# Autodesk Inventor assembly: COSI_MINI_V1
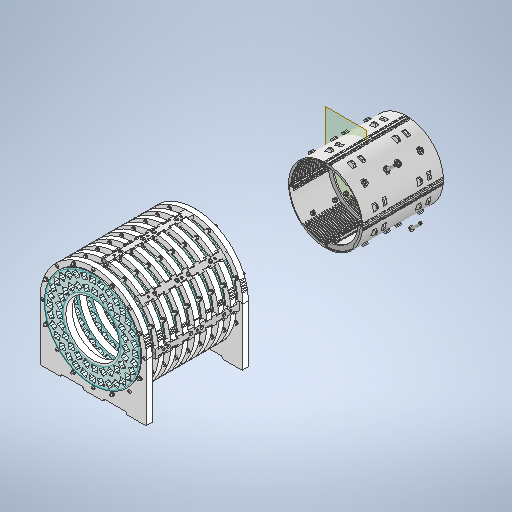
[picture p0: Inventor's stored thumbnail of the model, 512x512]
Saved by Autodesk Inventor 2025.2 (Build 292293000, 293)
## iProperties
Created: 2023-07-27
Part Number: COSI_MINI_V1
Document SubType Name: Assembly
Designer: Joshua Harper
Author: Joshua Harper
## Documents named in this file (17)
- C:\Users\Carla Fernandez\Documents\GitHub\OSII_MINI_V2\CAD MODELS\COSI_MINI_V2.iam
- C:\Users\Carla Fernandez\Documents\GitHub\OSII_MINI_V2\CAD MODELS\Ring_0.ipt
- C:\Users\Carla Fernandez\Documents\GitHub\OSII_MINI_V2\CAD MODELS\Ring_1.ipt
- C:\Users\Carla Fernandez\Documents\GitHub\OSII_MINI_V2\CAD MODELS\Ring_2.ipt
- C:\Users\Carla Fernandez\Documents\GitHub\OSII_MINI_V2\CAD MODELS\Ring_3.ipt
- C:\Users\Carla Fernandez\Documents\GitHub\OSII_MINI_V2\CAD MODELS\Ring_4.ipt
- C:\Users\Carla Fernandez\Documents\GitHub\OSII_MINI_V2\CAD MODELS\M4_threaded_brass.ipt
- C:\Users\Carla Fernandez\Documents\GitHub\OSII_MINI_V2\CAD MODELS\Locating_bar_V2.ipt
- C:\Users\Carla Fernandez\Documents\GitHub\OSII_MINI_V2\CAD MODELS\93187A150_NO THREADS_Brass Thin Hex Nut.ipt
- C:\Users\Carla Fernandez\Documents\GitHub\OSII_MINI_V2\CAD MODELS\98691A114_General Purpose Brass Washer.ipt
- C:\Users\Carla Fernandez\Documents\GitHub\OSII_MINI_V2\CAD MODELS\94500A283_NO THREADS_316 Stainless Steel Button Head Hex Drive Screws.ipt
- C:\Users\Carla Fernandez\Documents\GitHub\OSII_MINI_V2\CAD MODELS\94500A283_NO THREADS_316 Stainless Steel Button Head Hex Drive Screws_MIR.ipt
- C:\Users\Carla Fernandez\Documents\GitHub\OSII_MINI_V2\CAD MODELS\Lid_A.ipt
- C:\Users\Carla Fernandez\Documents\GitHub\OSII_MINI_V2\CAD MODELS\Lid_B.ipt
- C:\Users\Carla Fernandez\Documents\GitHub\OSII_MINI_V2\CAD MODELS\Shim_Assem_V4.iam
- C:\Users\Carla Fernandez\Documents\GitHub\OSII_MINI_V2\CAD MODELS\shim_cartridge_V3.ipt
- C:\Users\Carla Fernandez\Documents\GitHub\OSII_MINI_V2\CAD MODELS\shim_peg_V3.ipt
## Components (341 placed, 16 different names)
1. Ring_0:1 — Mate:4, Mate:5, Mate:16, Mate:37, Mate:39, Mate:43, Mate:48, Mate:51, Mate:54, Mate:55, Mate:57, Mate:70, Mate:71, Flush:3, Flush:4, Flush:5, Flush:6
2. Ring_1:1 — Mate:5, Mate:17, Flush:3
3. Ring_1:2 — Mate:3, Mate:4, Mate:10, Mate:16
4. Ring_2:1 — Mate:6, Mate:17, Flush:4
5. Ring_2:2 — Mate:2, Mate:3, Mate:9, Mate:10
6. Ring_3:1 — Mate:6, Mate:7, Flush:5
7. Ring_3:2 — Mate:1, Mate:2, Mate:8, Mate:9, Mate:36
8. Ring_4:1 — Mate:7, Flush:6, Mate:72, Mate:73
9. Ring_4:2 — Mate:1, Mate:8, Mate:26, Mate:35, Mate:62, Mate:63, Mate:68, Mate:76
10. Locating_bar_V2:1 — Mate:35, Mate:36, Mate:69
11. Locating_bar_V2:2 — Mate:37, Mate:39, Mate:76
12. Locating_bar_V2:3
13. Locating_bar_V2:4 — Mate:54
14. Locating_bar_V2:5 — Mate:43
15. Locating_bar_V2:6 — Mate:55, Mate:57
16. Locating_bar_V2:7 — Mate:51
17. Locating_bar_V2:8 — Mate:48
18. Shim_Assem_V4:1 [sub-assembly] — Mate:77, Mate:78, Mate:79, Mate:80, Mate:81
19. shim_cartridge_V3:1 — Mate:79, Mate:80, Mate:81
20. shim_peg_V3:1 — Mate:77, Mate:78
21. 94500A283_NO THREADS_316 Stainless Steel Button Head Hex Drive Screws:1 — Mate:68, Mate:69
22. 94500A283_NO THREADS_316 Stainless Steel Button Head Hex Drive Screws:2
23. 94500A283_NO THREADS_316 Stainless Steel Button Head Hex Drive Screws:3
24. 94500A283_NO THREADS_316 Stainless Steel Button Head Hex Drive Screws:4
25. 94500A283_NO THREADS_316 Stainless Steel Button Head Hex Drive Screws:5
26. 94500A283_NO THREADS_316 Stainless Steel Button Head Hex Drive Screws:6
27. 94500A283_NO THREADS_316 Stainless Steel Button Head Hex Drive Screws:7
28. 94500A283_NO THREADS_316 Stainless Steel Button Head Hex Drive Screws:8
29. Lid_A:1 — Mate:70, Mate:71
30. Lid_A:2
31. Lid_A:3
32. Lid_A:4
33. Lid_A:5
34. Lid_A:6
35. Lid_A:7
36. Lid_B:1
37. Lid_B:2
38. 94500A283_NO THREADS_316 Stainless Steel Button Head Hex Drive Screws_MIR:1 — Mate:72, Mate:73
39. 94500A283_NO THREADS_316 Stainless Steel Button Head Hex Drive Screws_MIR:2
40. 94500A283_NO THREADS_316 Stainless Steel Button Head Hex Drive Screws_MIR:3
41. 94500A283_NO THREADS_316 Stainless Steel Button Head Hex Drive Screws_MIR:4
42. 94500A283_NO THREADS_316 Stainless Steel Button Head Hex Drive Screws_MIR:5
43. 94500A283_NO THREADS_316 Stainless Steel Button Head Hex Drive Screws_MIR:6
44. 94500A283_NO THREADS_316 Stainless Steel Button Head Hex Drive Screws_MIR:7
45. 94500A283_NO THREADS_316 Stainless Steel Button Head Hex Drive Screws_MIR:8
46. M4_threaded_brass:1 — Mate:26
47. M4_threaded_brass:2
48. M4_threaded_brass:3
49. M4_threaded_brass:4
50. M4_threaded_brass:5
51. M4_threaded_brass:6
52. M4_threaded_brass:7
53. M4_threaded_brass:8
54. 93187A150_NO THREADS_Brass Thin Hex Nut:1 — Mate:67
55. 93187A150_NO THREADS_Brass Thin Hex Nut:2 — Mate:66
56. 98691A114_General Purpose Brass Washer:1 — Mate:62, Mate:67
57. 98691A114_General Purpose Brass Washer:2 — Mate:63, Mate:66
58. 93187A150_NO THREADS_Brass Thin Hex Nut:3
59. 93187A150_NO THREADS_Brass Thin Hex Nut:4
60. 98691A114_General Purpose Brass Washer:3
61. 98691A114_General Purpose Brass Washer:4
62. 93187A150_NO THREADS_Brass Thin Hex Nut:5
63. 93187A150_NO THREADS_Brass Thin Hex Nut:6
64. 98691A114_General Purpose Brass Washer:5
65. 98691A114_General Purpose Brass Washer:6
66. 93187A150_NO THREADS_Brass Thin Hex Nut:7
67. 93187A150_NO THREADS_Brass Thin Hex Nut:8
68. 98691A114_General Purpose Brass Washer:7
69. 98691A114_General Purpose Brass Washer:8
70. 93187A150_NO THREADS_Brass Thin Hex Nut:9
71. 93187A150_NO THREADS_Brass Thin Hex Nut:10
72. 98691A114_General Purpose Brass Washer:9
73. 98691A114_General Purpose Brass Washer:10
74. 93187A150_NO THREADS_Brass Thin Hex Nut:11
75. 93187A150_NO THREADS_Brass Thin Hex Nut:12
76. 98691A114_General Purpose Brass Washer:11
77. 98691A114_General Purpose Brass Washer:12
78. 93187A150_NO THREADS_Brass Thin Hex Nut:13
79. 93187A150_NO THREADS_Brass Thin Hex Nut:14
80. 98691A114_General Purpose Brass Washer:13
81. 98691A114_General Purpose Brass Washer:14
82. 93187A150_NO THREADS_Brass Thin Hex Nut:15
83. 93187A150_NO THREADS_Brass Thin Hex Nut:16
84. 98691A114_General Purpose Brass Washer:15
85. 98691A114_General Purpose Brass Washer:16
86. 93187A150_NO THREADS_Brass Thin Hex Nut:17
87. 93187A150_NO THREADS_Brass Thin Hex Nut:18
88. 98691A114_General Purpose Brass Washer:17
89. 98691A114_General Purpose Brass Washer:18
90. 93187A150_NO THREADS_Brass Thin Hex Nut:19
91. 93187A150_NO THREADS_Brass Thin Hex Nut:20
92. 98691A114_General Purpose Brass Washer:19
93. 98691A114_General Purpose Brass Washer:20
94. 93187A150_NO THREADS_Brass Thin Hex Nut:21
95. 93187A150_NO THREADS_Brass Thin Hex Nut:22
96. 98691A114_General Purpose Brass Washer:21
97. 98691A114_General Purpose Brass Washer:22
98. 93187A150_NO THREADS_Brass Thin Hex Nut:23
99. 93187A150_NO THREADS_Brass Thin Hex Nut:24
100. 98691A114_General Purpose Brass Washer:23
101. 98691A114_General Purpose Brass Washer:24
102. 93187A150_NO THREADS_Brass Thin Hex Nut:25
103. 93187A150_NO THREADS_Brass Thin Hex Nut:26
104. 98691A114_General Purpose Brass Washer:25
105. 98691A114_General Purpose Brass Washer:26
106. 93187A150_NO THREADS_Brass Thin Hex Nut:27
107. 93187A150_NO THREADS_Brass Thin Hex Nut:28
108. 98691A114_General Purpose Brass Washer:27
109. 98691A114_General Purpose Brass Washer:28
110. 93187A150_NO THREADS_Brass Thin Hex Nut:29
111. 93187A150_NO THREADS_Brass Thin Hex Nut:30
112. 98691A114_General Purpose Brass Washer:29
113. 98691A114_General Purpose Brass Washer:30
114. 93187A150_NO THREADS_Brass Thin Hex Nut:31
115. 93187A150_NO THREADS_Brass Thin Hex Nut:32
116. 98691A114_General Purpose Brass Washer:31
117. 98691A114_General Purpose Brass Washer:32
118. 93187A150_NO THREADS_Brass Thin Hex Nut:33
119. 93187A150_NO THREADS_Brass Thin Hex Nut:34
120. 98691A114_General Purpose Brass Washer:33
121. 98691A114_General Purpose Brass Washer:34
122. 93187A150_NO THREADS_Brass Thin Hex Nut:35
123. 93187A150_NO THREADS_Brass Thin Hex Nut:36
124. 98691A114_General Purpose Brass Washer:35
125. 98691A114_General Purpose Brass Washer:36
126. 93187A150_NO THREADS_Brass Thin Hex Nut:37
127. 93187A150_NO THREADS_Brass Thin Hex Nut:38
128. 98691A114_General Purpose Brass Washer:37
129. 98691A114_General Purpose Brass Washer:38
130. 93187A150_NO THREADS_Brass Thin Hex Nut:39
131. 93187A150_NO THREADS_Brass Thin Hex Nut:40
132. 98691A114_General Purpose Brass Washer:39
133. 98691A114_General Purpose Brass Washer:40
134. 93187A150_NO THREADS_Brass Thin Hex Nut:41
135. 93187A150_NO THREADS_Brass Thin Hex Nut:42
136. 98691A114_General Purpose Brass Washer:41
137. 98691A114_General Purpose Brass Washer:42
138. 93187A150_NO THREADS_Brass Thin Hex Nut:43
139. 93187A150_NO THREADS_Brass Thin Hex Nut:44
140. 98691A114_General Purpose Brass Washer:43
141. 98691A114_General Purpose Brass Washer:44
142. 93187A150_NO THREADS_Brass Thin Hex Nut:45
143. 93187A150_NO THREADS_Brass Thin Hex Nut:46
144. 98691A114_General Purpose Brass Washer:45
145. 98691A114_General Purpose Brass Washer:46
146. 93187A150_NO THREADS_Brass Thin Hex Nut:47
147. 93187A150_NO THREADS_Brass Thin Hex Nut:48
148. 98691A114_General Purpose Brass Washer:47
149. 98691A114_General Purpose Brass Washer:48
150. 93187A150_NO THREADS_Brass Thin Hex Nut:49
151. 93187A150_NO THREADS_Brass Thin Hex Nut:50
152. 98691A114_General Purpose Brass Washer:49
153. 98691A114_General Purpose Brass Washer:50
154. 93187A150_NO THREADS_Brass Thin Hex Nut:51
155. 93187A150_NO THREADS_Brass Thin Hex Nut:52
156. 98691A114_General Purpose Brass Washer:51
157. 98691A114_General Purpose Brass Washer:52
158. 93187A150_NO THREADS_Brass Thin Hex Nut:53
159. 93187A150_NO THREADS_Brass Thin Hex Nut:54
160. 98691A114_General Purpose Brass Washer:53
161. 98691A114_General Purpose Brass Washer:54
162. 93187A150_NO THREADS_Brass Thin Hex Nut:55
163. 93187A150_NO THREADS_Brass Thin Hex Nut:56
164. 98691A114_General Purpose Brass Washer:55
165. 98691A114_General Purpose Brass Washer:56
166. 93187A150_NO THREADS_Brass Thin Hex Nut:57
167. 93187A150_NO THREADS_Brass Thin Hex Nut:58
168. 98691A114_General Purpose Brass Washer:57
169. 98691A114_General Purpose Brass Washer:58
170. 93187A150_NO THREADS_Brass Thin Hex Nut:59
171. 93187A150_NO THREADS_Brass Thin Hex Nut:60
172. 98691A114_General Purpose Brass Washer:59
173. 98691A114_General Purpose Brass Washer:60
174. 93187A150_NO THREADS_Brass Thin Hex Nut:61
175. 93187A150_NO THREADS_Brass Thin Hex Nut:62
176. 98691A114_General Purpose Brass Washer:61
177. 98691A114_General Purpose Brass Washer:62
178. 93187A150_NO THREADS_Brass Thin Hex Nut:63
179. 93187A150_NO THREADS_Brass Thin Hex Nut:64
180. 98691A114_General Purpose Brass Washer:63
181. 98691A114_General Purpose Brass Washer:64
182. 93187A150_NO THREADS_Brass Thin Hex Nut:65
183. 93187A150_NO THREADS_Brass Thin Hex Nut:66
184. 98691A114_General Purpose Brass Washer:65
185. 98691A114_General Purpose Brass Washer:66
186. 93187A150_NO THREADS_Brass Thin Hex Nut:67
187. 93187A150_NO THREADS_Brass Thin Hex Nut:68
188. 98691A114_General Purpose Brass Washer:67
189. 98691A114_General Purpose Brass Washer:68
190. 93187A150_NO THREADS_Brass Thin Hex Nut:69
191. 93187A150_NO THREADS_Brass Thin Hex Nut:70
192. 98691A114_General Purpose Brass Washer:69
193. 98691A114_General Purpose Brass Washer:70
194. 93187A150_NO THREADS_Brass Thin Hex Nut:71
195. 93187A150_NO THREADS_Brass Thin Hex Nut:72
196. 98691A114_General Purpose Brass Washer:71
197. 98691A114_General Purpose Brass Washer:72
198. 93187A150_NO THREADS_Brass Thin Hex Nut:73
199. 93187A150_NO THREADS_Brass Thin Hex Nut:74
200. 98691A114_General Purpose Brass Washer:73
201. 98691A114_General Purpose Brass Washer:74
202. 93187A150_NO THREADS_Brass Thin Hex Nut:75
203. 93187A150_NO THREADS_Brass Thin Hex Nut:76
204. 98691A114_General Purpose Brass Washer:75
205. 98691A114_General Purpose Brass Washer:76
206. 93187A150_NO THREADS_Brass Thin Hex Nut:77
207. 93187A150_NO THREADS_Brass Thin Hex Nut:78
208. 98691A114_General Purpose Brass Washer:77
209. 98691A114_General Purpose Brass Washer:78
210. 93187A150_NO THREADS_Brass Thin Hex Nut:79
211. 93187A150_NO THREADS_Brass Thin Hex Nut:80
212. 98691A114_General Purpose Brass Washer:79
213. 98691A114_General Purpose Brass Washer:80
214. 93187A150_NO THREADS_Brass Thin Hex Nut:81
215. 93187A150_NO THREADS_Brass Thin Hex Nut:82
216. 98691A114_General Purpose Brass Washer:81
217. 98691A114_General Purpose Brass Washer:82
218. 93187A150_NO THREADS_Brass Thin Hex Nut:83
219. 93187A150_NO THREADS_Brass Thin Hex Nut:84
220. 98691A114_General Purpose Brass Washer:83
221. 98691A114_General Purpose Brass Washer:84
222. 93187A150_NO THREADS_Brass Thin Hex Nut:85
223. 93187A150_NO THREADS_Brass Thin Hex Nut:86
224. 98691A114_General Purpose Brass Washer:85
225. 98691A114_General Purpose Brass Washer:86
226. 93187A150_NO THREADS_Brass Thin Hex Nut:87
227. 93187A150_NO THREADS_Brass Thin Hex Nut:88
228. 98691A114_General Purpose Brass Washer:87
229. 98691A114_General Purpose Brass Washer:88
230. 93187A150_NO THREADS_Brass Thin Hex Nut:89
231. 93187A150_NO THREADS_Brass Thin Hex Nut:90
232. 98691A114_General Purpose Brass Washer:89
233. 98691A114_General Purpose Brass Washer:90
234. 93187A150_NO THREADS_Brass Thin Hex Nut:91
235. 93187A150_NO THREADS_Brass Thin Hex Nut:92
236. 98691A114_General Purpose Brass Washer:91
237. 98691A114_General Purpose Brass Washer:92
238. 93187A150_NO THREADS_Brass Thin Hex Nut:93
239. 93187A150_NO THREADS_Brass Thin Hex Nut:94
240. 98691A114_General Purpose Brass Washer:93
241. 98691A114_General Purpose Brass Washer:94
242. 93187A150_NO THREADS_Brass Thin Hex Nut:95
243. 93187A150_NO THREADS_Brass Thin Hex Nut:96
244. 98691A114_General Purpose Brass Washer:95
245. 98691A114_General Purpose Brass Washer:96
246. 93187A150_NO THREADS_Brass Thin Hex Nut:97
247. 93187A150_NO THREADS_Brass Thin Hex Nut:98
248. 98691A114_General Purpose Brass Washer:97
249. 98691A114_General Purpose Brass Washer:98
250. 93187A150_NO THREADS_Brass Thin Hex Nut:99
251. 93187A150_NO THREADS_Brass Thin Hex Nut:100
252. 98691A114_General Purpose Brass Washer:99
253. 98691A114_General Purpose Brass Washer:100
254. 93187A150_NO THREADS_Brass Thin Hex Nut:101
255. 93187A150_NO THREADS_Brass Thin Hex Nut:102
256. 98691A114_General Purpose Brass Washer:101
257. 98691A114_General Purpose Brass Washer:102
258. 93187A150_NO THREADS_Brass Thin Hex Nut:103
259. 93187A150_NO THREADS_Brass Thin Hex Nut:104
260. 98691A114_General Purpose Brass Washer:103
261. 98691A114_General Purpose Brass Washer:104
262. 93187A150_NO THREADS_Brass Thin Hex Nut:105
263. 93187A150_NO THREADS_Brass Thin Hex Nut:106
264. 98691A114_General Purpose Brass Washer:105
265. 98691A114_General Purpose Brass Washer:106
266. 93187A150_NO THREADS_Brass Thin Hex Nut:107
267. 93187A150_NO THREADS_Brass Thin Hex Nut:108
268. 98691A114_General Purpose Brass Washer:107
269. 98691A114_General Purpose Brass Washer:108
270. 93187A150_NO THREADS_Brass Thin Hex Nut:109
271. 93187A150_NO THREADS_Brass Thin Hex Nut:110
272. 98691A114_General Purpose Brass Washer:109
273. 98691A114_General Purpose Brass Washer:110
274. 93187A150_NO THREADS_Brass Thin Hex Nut:111
275. 93187A150_NO THREADS_Brass Thin Hex Nut:112
276. 98691A114_General Purpose Brass Washer:111
277. 98691A114_General Purpose Brass Washer:112
278. 93187A150_NO THREADS_Brass Thin Hex Nut:113
279. 93187A150_NO THREADS_Brass Thin Hex Nut:114
280. 98691A114_General Purpose Brass Washer:113
281. 98691A114_General Purpose Brass Washer:114
282. 93187A150_NO THREADS_Brass Thin Hex Nut:115
283. 93187A150_NO THREADS_Brass Thin Hex Nut:116
284. 98691A114_General Purpose Brass Washer:115
285. 98691A114_General Purpose Brass Washer:116
286. 93187A150_NO THREADS_Brass Thin Hex Nut:117
287. 93187A150_NO THREADS_Brass Thin Hex Nut:118
288. 98691A114_General Purpose Brass Washer:117
289. 98691A114_General Purpose Brass Washer:118
290. 93187A150_NO THREADS_Brass Thin Hex Nut:119
291. 93187A150_NO THREADS_Brass Thin Hex Nut:120
292. 98691A114_General Purpose Brass Washer:119
293. 98691A114_General Purpose Brass Washer:120
294. 93187A150_NO THREADS_Brass Thin Hex Nut:121
295. 93187A150_NO THREADS_Brass Thin Hex Nut:122
296. 98691A114_General Purpose Brass Washer:121
297. 98691A114_General Purpose Brass Washer:122
298. 93187A150_NO THREADS_Brass Thin Hex Nut:123
299. 93187A150_NO THREADS_Brass Thin Hex Nut:124
300. 98691A114_General Purpose Brass Washer:123
301. 98691A114_General Purpose Brass Washer:124
302. 93187A150_NO THREADS_Brass Thin Hex Nut:125
303. 93187A150_NO THREADS_Brass Thin Hex Nut:126
304. 98691A114_General Purpose Brass Washer:125
305. 98691A114_General Purpose Brass Washer:126
306. 93187A150_NO THREADS_Brass Thin Hex Nut:127
307. 93187A150_NO THREADS_Brass Thin Hex Nut:128
308. 98691A114_General Purpose Brass Washer:127
309. 98691A114_General Purpose Brass Washer:128
310. 93187A150_NO THREADS_Brass Thin Hex Nut:129
311. 93187A150_NO THREADS_Brass Thin Hex Nut:130
312. 98691A114_General Purpose Brass Washer:129
313. 98691A114_General Purpose Brass Washer:130
314. 93187A150_NO THREADS_Brass Thin Hex Nut:131
315. 93187A150_NO THREADS_Brass Thin Hex Nut:132
316. 98691A114_General Purpose Brass Washer:131
317. 98691A114_General Purpose Brass Washer:132
318. 93187A150_NO THREADS_Brass Thin Hex Nut:133
319. 93187A150_NO THREADS_Brass Thin Hex Nut:134
320. 98691A114_General Purpose Brass Washer:133
321. 98691A114_General Purpose Brass Washer:134
322. 93187A150_NO THREADS_Brass Thin Hex Nut:135
323. 93187A150_NO THREADS_Brass Thin Hex Nut:136
324. 98691A114_General Purpose Brass Washer:135
325. 98691A114_General Purpose Brass Washer:136
326. 93187A150_NO THREADS_Brass Thin Hex Nut:137
327. 93187A150_NO THREADS_Brass Thin Hex Nut:138
328. 98691A114_General Purpose Brass Washer:137
329. 98691A114_General Purpose Brass Washer:138
330. 93187A150_NO THREADS_Brass Thin Hex Nut:139
331. 93187A150_NO THREADS_Brass Thin Hex Nut:140
332. 98691A114_General Purpose Brass Washer:139
333. 98691A114_General Purpose Brass Washer:140
334. 93187A150_NO THREADS_Brass Thin Hex Nut:141
335. 93187A150_NO THREADS_Brass Thin Hex Nut:142
336. 98691A114_General Purpose Brass Washer:141
337. 98691A114_General Purpose Brass Washer:142
338. 93187A150_NO THREADS_Brass Thin Hex Nut:143
339. 93187A150_NO THREADS_Brass Thin Hex Nut:144
340. 98691A114_General Purpose Brass Washer:143
341. 98691A114_General Purpose Brass Washer:144
## Component patterns: (8 elements), (8 elements, first: 94500A283_NO THREADS_316 Stainless Steel Button Head Hex Drive Screws:1), (7 elements, first: Lid_A:1), (2 elements, first: Lid_B:1), (8 elements, first: 94500A283_NO THREADS_316 Stainless Steel Button Head Hex Drive Screws_MIR:1), (8 elements, first: M4_threaded_brass:1), (9 elements, first: 93187A150_NO THREADS_Brass Thin Hex Nut:1 + 93187A150_NO THREADS_Brass Thin Hex Nut:2 + 98691A114_General Purpose Brass Washer:1 + 98691A114_General Purpose Brass Washer:2), Component Pattern 1:2 (9 elements), Component Pattern 1:3 (9 elements), Component Pattern 1:4 (9 elements), Component Pattern 1:5 (9 elements), Component Pattern 1:6 (9 elements), Component Pattern 1:7 (9 elements), Component Pattern 1:8 (9 elements)
## Relationships (43: Mate 39, Flush 4)
- Mate:1 (13 mm): Ring_3:2 ↔ Ring_4:2
- Mate:2 (13 mm): Ring_2:2 ↔ Ring_3:2
- Mate:3 (13 mm): Ring_1:2 ↔ Ring_2:2
- Mate:4 (13 mm): Ring_0:1 ↔ Ring_1:2
- Mate:5 (13 mm): Ring_0:1 ↔ Ring_1:1
- Mate:6 (13 mm): Ring_2:1 ↔ Ring_3:1
- Mate:7 (13 mm): Ring_3:1 ↔ Ring_4:1
- Mate:8: Ring_3:2 ↔ Ring_4:2
- Mate:9: Ring_2:2 ↔ Ring_3:2
- Mate:10: Ring_1:2 ↔ Ring_2:2
- Mate:16: Ring_0:1 ↔ Ring_1:2
- Mate:17 (13 mm): Ring_1:1 ↔ Ring_2:1
- Mate:26: Ring_4:2 ↔ M4_threaded_brass:1
- Mate:35: Ring_4:2 ↔ Locating_bar_V2:1
- Mate:36: Ring_3:2 ↔ Locating_bar_V2:1
- Mate:37: Ring_0:1 ↔ Locating_bar_V2:2
- Mate:39: Ring_0:1 ↔ Locating_bar_V2:2
- Mate:43: Ring_0:1 ↔ Locating_bar_V2:5
- Mate:48: Ring_0:1 ↔ Locating_bar_V2:8
- Mate:51: Ring_0:1 ↔ Locating_bar_V2:7
- Mate:54: Ring_0:1 ↔ Locating_bar_V2:4
- Mate:55: Ring_0:1 ↔ Locating_bar_V2:6
- Mate:57: Ring_0:1 ↔ Locating_bar_V2:6
- Mate:62: Ring_4:2 ↔ 98691A114_General Purpose Brass Washer:1
- Mate:63: Ring_4:2 ↔ 98691A114_General Purpose Brass Washer:2
- Mate:66: 93187A150_NO THREADS_Brass Thin Hex Nut:2 ↔ 98691A114_General Purpose Brass Washer:2
- Mate:67: 93187A150_NO THREADS_Brass Thin Hex Nut:1 ↔ 98691A114_General Purpose Brass Washer:1
- Mate:68: Ring_4:2 ↔ 94500A283_NO THREADS_316 Stainless Steel Button Head Hex Drive Screws:1
- Mate:69: Locating_bar_V2:1 ↔ 94500A283_NO THREADS_316 Stainless Steel Button Head Hex Drive Screws:1
- Mate:70 (0.5 mm): Ring_0:1 ↔ Lid_A:1
- Mate:71: Ring_0:1 ↔ Lid_A:1
- Flush:3: Ring_0:1 ↔ Ring_1:1
- Flush:4: Ring_0:1 ↔ Ring_2:1
- Flush:5: Ring_0:1 ↔ Ring_3:1
- Flush:6: Ring_0:1 ↔ Ring_4:1
- Mate:72: Ring_4:1 ↔ 94500A283_NO THREADS_316 Stainless Steel Button Head Hex Drive Screws_MIR:1
- Mate:73: Ring_4:1 ↔ 94500A283_NO THREADS_316 Stainless Steel Button Head Hex Drive Screws_MIR:1
- Mate:76: Ring_4:2 ↔ Locating_bar_V2:2
- Mate:77: Shim_Assem_V4:1 ↔ shim_peg_V3:1
- Mate:78: Shim_Assem_V4:1 ↔ shim_peg_V3:1
- Mate:79: Shim_Assem_V4:1 ↔ shim_cartridge_V3:1
- Mate:80: Shim_Assem_V4:1 ↔ shim_cartridge_V3:1
- Mate:81: Shim_Assem_V4:1 ↔ shim_cartridge_V3:1
